# Autodesk Inventor assembly: GFRP_T3_02
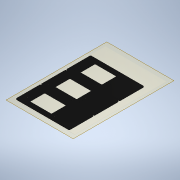
[picture p0: Inventor's stored thumbnail of the model, 180x180]
Saved by Autodesk Inventor 2020 (Build 240168000, 168)
## iProperties
Created: 2021-08-27
Part Number: GFRP_T3_02
Document SubType Name: Assembly
Designer: Masato
Author: Masato
## Documents named in this file (3)
- C:\Inventor\SUSTAINA-OP\Cam\GFRP_T3_02.iam
- C:\Inventor\SUSTAINA-OP\Cam\DisposableBoard.ipt
- C:\Inventor\SUSTAINA-OP\LowerBody\Foot\Sole_frame.ipt
## Components (4 placed, 2 different names)
1. DisposableBoard:1 — メイト:2, メイト:1, フラッシュ:1, フラッシュ:2, メイト:4, メイト:5, メイト:6, フラッシュ:3, フラッシュ:4
2. Sole_frame:1 — メイト:4, フラッシュ:3, フラッシュ:4, フラッシュ:5, メイト:7
3. Sole_frame:2 — メイト:5, フラッシュ:5, メイト:7, フラッシュ:6, メイト:8
4. Sole_frame:3 — メイト:6, フラッシュ:6, メイト:8
## Relationships (13: Mate 7, Flush 6)
- メイト:2 [Mate]: DisposableBoard:1
- メイト:1 [Mate]: DisposableBoard:1
- フラッシュ:1 [Flush]: DisposableBoard:1
- フラッシュ:2 [Flush]: DisposableBoard:1
- メイト:4 [Mate]: DisposableBoard:1 ↔ Sole_frame:1
- メイト:5 [Mate]: DisposableBoard:1 ↔ Sole_frame:2
- メイト:6 [Mate]: DisposableBoard:1 ↔ Sole_frame:3
- フラッシュ:3 [Flush] (2.5 mm): DisposableBoard:1 ↔ Sole_frame:1
- フラッシュ:4 [Flush] (4.5 mm): DisposableBoard:1 ↔ Sole_frame:1
- フラッシュ:5 [Flush]: Sole_frame:1 ↔ Sole_frame:2
- メイト:7 [Mate] (2.5 mm): Sole_frame:1 ↔ Sole_frame:2
- フラッシュ:6 [Flush]: Sole_frame:2 ↔ Sole_frame:3
- メイト:8 [Mate] (2.5 mm): Sole_frame:2 ↔ Sole_frame:3
